# Autodesk Inventor assembly: Ensamble_del_hexapod_V1
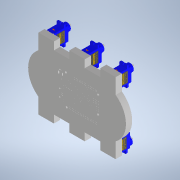
[picture p0: Inventor's stored thumbnail of the model, 180x180]
Saved by Autodesk Inventor 2021 (Build 250183000, 183)
## iProperties
Created: 2021-02-17
Part Number: Ensamble_del_hexapod_V1
Document SubType Name: Assembly
Designer: Admin
Author: Admin
## Documents named in this file (4)
- C:\Users\Admin\Documents\UVG\Semestre 10\Robotica 1\Proyecto de Robot Hexapodo\Proyecto_de_Hexapod_GP_RF\Ensamble_del_hexapod_V1.iam
- C:\Users\Admin\Documents\UVG\Semestre 10\Robotica 1\Proyecto de Robot Hexapodo\Proyecto_de_Hexapod_GP_RF\SG90 - Micro Servo 9g - Tower Pro.iam
- C:\Users\Admin\Documents\UVG\Semestre 10\Robotica 1\Proyecto de Robot Hexapodo\Proyecto_de_Hexapod_GP_RF\Arduino UNO Rev.3 (CH340)-CAWEB.ORG.iam
- C:\Users\Admin\Documents\UVG\Semestre 10\Robotica 1\Proyecto de Robot Hexapodo\Proyecto_de_Hexapod_GP_RF\Base Para Arduino y Servos.ipt
## Components (8 placed, 3 different names)
1. Arduino UNO Rev.3 (CH340)-CAWEB.ORG:1 [sub-assembly] — Flush:1
2. SG90 - Micro Servo 9g - Tower Pro:1 [sub-assembly] — Mate:2
3. SG90 - Micro Servo 9g - Tower Pro:2 [sub-assembly] — Mate:1
4. SG90 - Micro Servo 9g - Tower Pro:3 [sub-assembly] — Mate:3
5. SG90 - Micro Servo 9g - Tower Pro:4 [sub-assembly] — Mate:4
6. Base Para Arduino y Servos:1 — Flush:1, Mate:1, Mate:2, Mate:3, Mate:4, Mate:5, Mate:6
7. SG90 - Micro Servo 9g - Tower Pro:5 [sub-assembly] — Mate:6
8. SG90 - Micro Servo 9g - Tower Pro:6 [sub-assembly] — Mate:5
## Relationships (7: Mate 6, Flush 1)
- Flush:1: Arduino UNO Rev.3 (CH340)-CAWEB.ORG:1 ↔ Base Para Arduino y Servos:1
- Mate:1: SG90 - Micro Servo 9g - Tower Pro:2 ↔ Base Para Arduino y Servos:1
- Mate:2: SG90 - Micro Servo 9g - Tower Pro:1 ↔ Base Para Arduino y Servos:1
- Mate:3: SG90 - Micro Servo 9g - Tower Pro:3 ↔ Base Para Arduino y Servos:1
- Mate:4: SG90 - Micro Servo 9g - Tower Pro:4 ↔ Base Para Arduino y Servos:1
- Mate:5: Base Para Arduino y Servos:1 ↔ SG90 - Micro Servo 9g - Tower Pro:6
- Mate:6: Base Para Arduino y Servos:1 ↔ SG90 - Micro Servo 9g - Tower Pro:5
